# Autodesk Inventor assembly: SE. fuente
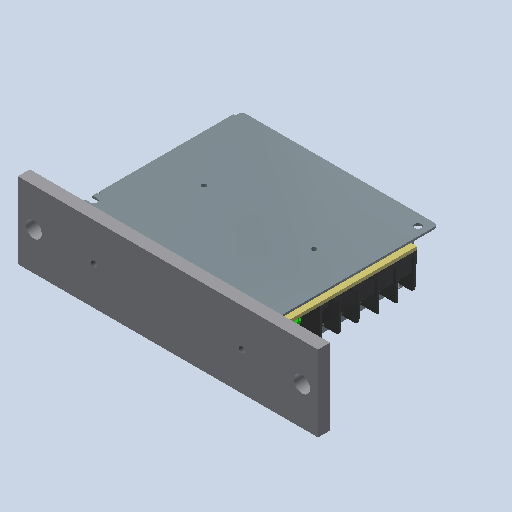
[picture p0: Inventor's stored thumbnail of the model, 512x512]
Saved by Autodesk Inventor 2024.2 (Build 282272000, 272)
## iProperties
Created: 2025-06-19
Part Number: SE. fuente
Material: Genérico
Document SubType Name: Assembly
Designer: jd.castellanosq
Author: jd.castellanosq
## Documents named in this file (3)
- I:\MICROMECANICA\ALTAS ENERGIAS\Deteccion de Muones\Detectores centelladores\Partes Detectores centelladores\Chasis DC\Partes Chasis DC\SE. fuente.iam
- I:\MICROMECANICA\ALTAS ENERGIAS\Deteccion de Muones\Detectores centelladores\Partes Detectores centelladores\Chasis DC\Partes Chasis DC\Soporte fuente.ipt
- I:\MICROMECANICA\ALTAS ENERGIAS\Deteccion de Muones\Detectores centelladores\Partes Detectores centelladores\PARTES DC\Tarjetas IC DC\LRS-50-Series(MW)\LRS-50-Series(MW).ipt
## Components (2 placed, 2 different names)
1. Soporte fuente:1 — Coincidencia:1, Nivelación:1, Coincidencia:2, Coincidencia:3, Coincidencia:4, Coincidencia:5
2. LRS-50-Series(MW):1 — Coincidencia:3, Coincidencia:4, Coincidencia:5
## Relationships (6: Mate 5, Flush 1)
- Coincidencia:1 [Mate]: Soporte fuente:1
- Nivelación:1 [Flush]: Soporte fuente:1
- Coincidencia:2 [Mate]: Soporte fuente:1
- Coincidencia:3 [Mate]: Soporte fuente:1 ↔ LRS-50-Series(MW):1
- Coincidencia:4 [Mate]: Soporte fuente:1 ↔ LRS-50-Series(MW):1
- Coincidencia:5 [Mate]: Soporte fuente:1 ↔ LRS-50-Series(MW):1
